# Autodesk Inventor assembly: ASY TZS 1410 charging hatch
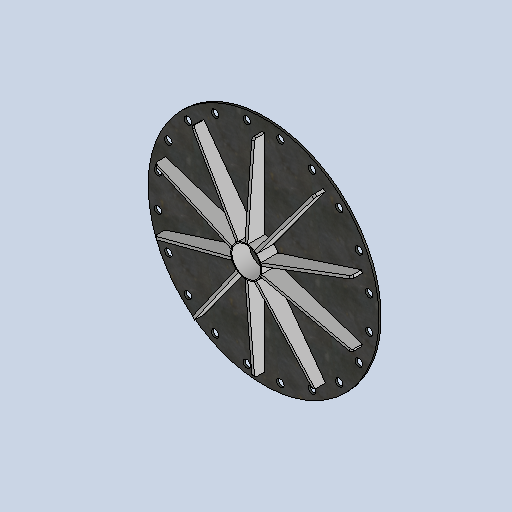
[picture p0: Inventor's stored thumbnail of the model, 512x512]
Saved by Autodesk Inventor 2025 (Build 290162010, 162A)
## iProperties
Created: 2025-04-22
Part Number: ASY TZS 1410 charging hatch
Document SubType Name: Assembly
Designer: user
Author: user
## Documents named in this file (4)
- C:\Users\pokla\Documents\Inventor\TZS-Tazovskiy\ASY TZS 1410 charging hatch.iam
- C:\Users\pokla\Documents\Inventor\TZS-Tazovskiy\TZS 1412 charging hatch 500mm.ipt
- C:\Users\pokla\Documents\Inventor\TZS-Tazovskiy\TZS 1413 charging hatch reinf.ipt
- C:\Users\pokla\Documents\Inventor\TZS-Tazovskiy\TZS 1411 hatch tube 500mm.ipt
## Components (12 placed, 3 different names)
1. APN 1412 charging hatch 500mm.ipt:1 — Rigid:1, Flush:1
2. APN 1411 hatch tube 500mm.ipt:1 — Rigid:1
3. APN 1413 charging hatch reinf.ipt:1 — Mate:1, Flush:1, Mate:2, Mate:3
4. APN 1413 charging hatch reinf.ipt:2
5. APN 1413 charging hatch reinf.ipt:3
6. APN 1413 charging hatch reinf.ipt:4
7. APN 1413 charging hatch reinf.ipt:5
8. APN 1413 charging hatch reinf.ipt:6
9. APN 1413 charging hatch reinf.ipt:7
10. APN 1413 charging hatch reinf.ipt:8
11. APN 1413 charging hatch reinf.ipt:9
12. APN 1413 charging hatch reinf.ipt:10
## Component patterns: (10 elements, first: APN 1413 charging hatch reinf.ipt:1)
## Relationships (5: Mate 3, WeldJoint 1, Flush 1)
- Rigid:1 [WeldJoint]: APN 1412 charging hatch 500mm.ipt:1 ↔ APN 1411 hatch tube 500mm.ipt:1
- Mate:1: APN 1413 charging hatch reinf.ipt:1
- Flush:1: APN 1412 charging hatch 500mm.ipt:1 ↔ APN 1413 charging hatch reinf.ipt:1
- Mate:2: APN 1413 charging hatch reinf.ipt:1
- Mate:3: APN 1413 charging hatch reinf.ipt:1
